# Autodesk Inventor assembly: SuspensionFinalShowdown
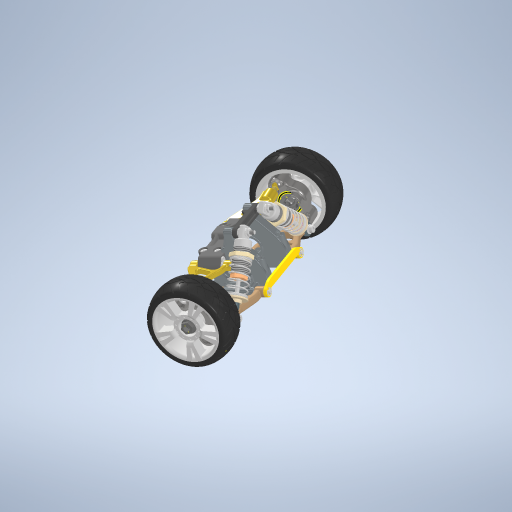
[picture p0: Inventor's stored thumbnail of the model, 512x512]
Saved by Autodesk Inventor 2024 (Build 280153000, 153)
## iProperties
Created: 2023-07-07
Part Number: SuspensionFinalShowdown
Document SubType Name: Assembly
Designer: birud
Author: birud
## Documents named in this file (20)
- C:\Users\_Astitva_Aryan_\Downloads\ES101_Components_Group5\Suspension_Final_Assembly.iam
- C:\Users\_Astitva_Aryan_\Downloads\ES101_Components_Group5\Components_derived\Front side plate L-1.ipt
- C:\Users\_Astitva_Aryan_\Downloads\ES101_Components_Group5\Components_derived\Front side plate R-1.ipt
- C:\Users\_Astitva_Aryan_\Downloads\ES101_Components_Group5\Components_derived\Front upper mount.ipt
- C:\Users\_Astitva_Aryan_\Downloads\ES101_Components_Group5\Components_derived\Front Shock Brace-1.ipt
- C:\Users\_Astitva_Aryan_\Downloads\ES101_Components_Group5\Components_derived\Front Lower arm Brace.ipt
- C:\Users\_Astitva_Aryan_\Downloads\ES101_Components_Group5\Components_derived\Front Lower Hinge Pin.ipt
- C:\Users\_Astitva_Aryan_\Downloads\ES101_Components_Group5\Components_derived\Front Upper Hinge Pin.ipt
- C:\Users\_Astitva_Aryan_\Downloads\ES101_Components_Group5\Components_derived\Front Upper Arm with pillow ball.iam
- C:\Users\_Astitva_Aryan_\Downloads\ES101_Components_Group5\Components_derived\Front Lower Arm with pillow ball.iam
- C:\Users\_Astitva_Aryan_\Downloads\ES101_Components_Group5\Components_derived\Shock Bushing.ipt
- C:\Users\_Astitva_Aryan_\Downloads\ES101_Components_Group5\Components_derived\Front Suspension Adjustment Clip.ipt
- C:\Users\_Astitva_Aryan_\Downloads\ES101_Components_Group5\Components_derived\a shock absorber.iam
- C:\Users\_Astitva_Aryan_\Downloads\ES101_Components_Group5\Components_derived\Front Hub Carrier L.iam
- C:\Users\_Astitva_Aryan_\Downloads\ES101_Components_Group5\Components_derived\SA E-Clip.ipt
- C:\Users\_Astitva_Aryan_\Downloads\ES101_Components_Group5\Components_derived\ANSI B18.22.1 - No. 5.ipt
- C:\Users\_Astitva_Aryan_\Downloads\ES101_Components_Group5\Components_derived\P12.ipt
- C:\Users\_Astitva_Aryan_\Downloads\ES101_Components_Group5\Components_derived\P20.ipt
- C:\Users\_Astitva_Aryan_\Downloads\ES101_Components_Group5\Components_derived\P20-nut.ipt
- C:\Users\_Astitva_Aryan_\Downloads\ES101_Components_Group5\Components_derived\Front Hub Carrier R.iam
## Components (43 placed, 19 different names)
1. Front side plate L-1:1 — Mate:1, Flush:1, Mate:2, Mate:4, Mate:5, Mate:6, Mate:7, Mate:12, Mate:50, Mate:52, Insert:11
2. Front side plate R-1:1 — Mate:1, Flush:1, Mate:2, Mate:3, Mate:8, Mate:9, Mate:11, Mate:21, Mate:22, Insert:12
3. Front upper mount:1 — Mate:3, Mate:4, Mate:5, Mate:14, Mate:15, Mate:24, Mate:26, Mate:42, Mate:47, Mate:48, Insert:5, Insert:6, Insert:7, Insert:8
4. Front Shock Brace-1:1 — Mate:6, Mate:7, Mate:8, Mate:17, Mate:18, Mate:19, Mate:20
5. Front Lower arm Brace:1 — Mate:9, Flush:4, Mate:51
6. Front Lower Hinge Pin:1 — Mate:12, Flush:2, Mate:49
7. Front Lower Hinge Pin:2 — Mate:11, Flush:2, Mate:33, Mate:34, Flush:4, Mate:35
8. Front Upper Hinge Pin:1 — Mate:15, Flush:3, Mate:23, Mate:37, Mate:38, Flush:5, Mate:39, Mate:40
9. Front Upper Hinge Pin:2 — Mate:14, Flush:3, Mate:41, Mate:43, Mate:44, Mate:45
10. Front Lower Arm with pillow ball:1 [sub-assembly] — Mate:21, Mate:22, Mate:29, Mate:32, Mate:36
11. Shock Bushing:1 — Mate:17, Mate:18, Mate:28, Mate:30, Insert:2
12. Shock Bushing:2 — Mate:19, Mate:20, Mate:56, Mate:58, Insert:4
13. Front Upper Arm with pillow ball:1 [sub-assembly] — Mate:23, Mate:24, Mate:27, Mate:31, Flush:5
14. Front Suspension Adjustment Clip:1 — Mate:26, Mate:27
15. a shock absorber:1 [sub-assembly] — Mate:28, Mate:29, Mate:30, Insert:1, Insert:10
16. Front Hub Carrier L:1 [sub-assembly] — Mate:31, Mate:32
17. SA E-Clip:1 — Mate:33, Mate:34
18. SA E-Clip:2 — Mate:35, Mate:36
19. SA E-Clip:3 — Mate:37, Mate:38
20. SA E-Clip:4 — Mate:39, Mate:40
21. ANSI B18.22.1 - No. 5:1 — Insert:1
22. ANSI B18.22.1 - No. 5:2 — Insert:2, Mate:60
23. Front Upper Arm with pillow ball:2 [sub-assembly] — Mate:41, Mate:42, Mate:46, Mate:63
24. SA E-Clip:5 — Mate:43, Mate:44
25. SA E-Clip:6 — Mate:45, Mate:46
26. Front Suspension Adjustment Clip:2 — Mate:47, Mate:48
27. Front Lower Arm with pillow ball:2 [sub-assembly] — Mate:49, Mate:50, Mate:54, Mate:55, Mate:57, Mate:64
28. SA E-Clip:7 — Mate:51, Mate:52
29. SA E-Clip:8 — Mate:54, Mate:55
30. a shock absorber:2 [sub-assembly] — Mate:56, Mate:57, Mate:58, Insert:3, Insert:9
31. ANSI B18.22.1 - No. 5:3 — Insert:3
32. ANSI B18.22.1 - No. 5:4 — Insert:4, Mate:61
33. P12:1 — Insert:5
34. P12:2 — Insert:8
35. P12:3 — Insert:7
36. P12:4 — Insert:6
37. P12:5 — Insert:9
38. P12:6 — Insert:10
39. P20:1 — Insert:12, Mate:59
40. P20:2 — Insert:11, Mate:62
41. P20-nut:1 — Mate:59, Mate:60
42. P20-nut:2 — Mate:61, Mate:62
43. Front Hub Carrier R:1 [sub-assembly] — Mate:63, Mate:64
## Relationships (76: Mate 59, Insert 12, Flush 5)
- Mate:1: Front side plate L-1:1 ↔ Front side plate R-1:1
- Flush:1: Front side plate L-1:1 ↔ Front side plate R-1:1
- Mate:2 (251.46 mm): Front side plate L-1:1 ↔ Front side plate R-1:1
- Mate:3: Front side plate R-1:1 ↔ Front upper mount:1
- Mate:4: Front side plate L-1:1 ↔ Front upper mount:1
- Mate:5: Front side plate L-1:1 ↔ Front upper mount:1
- Mate:6: Front side plate L-1:1 ↔ Front Shock Brace-1:1
- Mate:7: Front side plate L-1:1 ↔ Front Shock Brace-1:1
- Mate:8: Front side plate R-1:1 ↔ Front Shock Brace-1:1
- Mate:9: Front side plate R-1:1 ↔ Front Lower arm Brace:1
- Mate:11: Front side plate R-1:1 ↔ Front Lower Hinge Pin:2
- Mate:12: Front side plate L-1:1 ↔ Front Lower Hinge Pin:1
- Flush:2: Front Lower Hinge Pin:1 ↔ Front Lower Hinge Pin:2
- Mate:14: Front upper mount:1 ↔ Front Upper Hinge Pin:2
- Mate:15: Front upper mount:1 ↔ Front Upper Hinge Pin:1
- Flush:3: Front Upper Hinge Pin:1 ↔ Front Upper Hinge Pin:2
- Mate:17: Front Shock Brace-1:1 ↔ Shock Bushing:1
- Mate:18: Front Shock Brace-1:1 ↔ Shock Bushing:1
- Mate:19: Front Shock Brace-1:1 ↔ Shock Bushing:2
- Mate:20: Front Shock Brace-1:1 ↔ Shock Bushing:2
- Mate:21: Front side plate R-1:1 ↔ Front Lower Arm with pillow ball:1
- Mate:22: Front side plate R-1:1 ↔ Front Lower Arm with pillow ball:1
- Mate:23: Front Upper Hinge Pin:1 ↔ Front Upper Arm with pillow ball:1
- Mate:24: Front upper mount:1 ↔ Front Upper Arm with pillow ball:1
- Mate:26: Front upper mount:1 ↔ Front Suspension Adjustment Clip:1
- Mate:27: Front Upper Arm with pillow ball:1 ↔ Front Suspension Adjustment Clip:1
- Mate:28: Shock Bushing:1 ↔ a shock absorber:1
- Mate:29: Front Lower Arm with pillow ball:1 ↔ a shock absorber:1
- Mate:30: Shock Bushing:1 ↔ a shock absorber:1
- Mate:31: Front Upper Arm with pillow ball:1 ↔ Front Hub Carrier L:1
- Mate:32: Front Lower Arm with pillow ball:1 ↔ Front Hub Carrier L:1
- Mate:33: Front Lower Hinge Pin:2 ↔ SA E-Clip:1
- Mate:34: Front Lower Hinge Pin:2 ↔ SA E-Clip:1
- Flush:4: Front Lower arm Brace:1 ↔ Front Lower Hinge Pin:2
- Mate:35: Front Lower Hinge Pin:2 ↔ SA E-Clip:2
- Mate:36: Front Lower Arm with pillow ball:1 ↔ SA E-Clip:2
- Mate:37: Front Upper Hinge Pin:1 ↔ SA E-Clip:3
- Mate:38: Front Upper Hinge Pin:1 ↔ SA E-Clip:3
- Flush:5: Front Upper Hinge Pin:1 ↔ Front Upper Arm with pillow ball:1
- Mate:39: Front Upper Hinge Pin:1 ↔ SA E-Clip:4
- Mate:40: Front Upper Hinge Pin:1 ↔ SA E-Clip:4
- Insert:1: a shock absorber:1 ↔ ANSI B18.22.1 - No. 5:1
- Insert:2: Shock Bushing:1 ↔ ANSI B18.22.1 - No. 5:2
- Mate:41: Front Upper Hinge Pin:2 ↔ Front Upper Arm with pillow ball:2
- Mate:42: Front upper mount:1 ↔ Front Upper Arm with pillow ball:2
- Mate:43: Front Upper Hinge Pin:2 ↔ SA E-Clip:5
- Mate:44: Front Upper Hinge Pin:2 ↔ SA E-Clip:5
- Mate:45: Front Upper Hinge Pin:2 ↔ SA E-Clip:6
- Mate:46: Front Upper Arm with pillow ball:2 ↔ SA E-Clip:6
- Mate:47: Front upper mount:1 ↔ Front Suspension Adjustment Clip:2
- Mate:48: Front upper mount:1 ↔ Front Suspension Adjustment Clip:2
- Mate:49: Front Lower Hinge Pin:1 ↔ Front Lower Arm with pillow ball:2
- Mate:50: Front side plate L-1:1 ↔ Front Lower Arm with pillow ball:2
- Mate:51: Front Lower arm Brace:1 ↔ SA E-Clip:7
- Mate:52: Front side plate L-1:1 ↔ SA E-Clip:7
- Mate:54: Front Lower Arm with pillow ball:2 ↔ SA E-Clip:8
- Mate:55: Front Lower Arm with pillow ball:2 ↔ SA E-Clip:8
- Mate:56: Shock Bushing:2 ↔ a shock absorber:2
- Mate:57: Front Lower Arm with pillow ball:2 ↔ a shock absorber:2
- Mate:58: Shock Bushing:2 ↔ a shock absorber:2
- Insert:3: a shock absorber:2 ↔ ANSI B18.22.1 - No. 5:3
- Insert:4: Shock Bushing:2 ↔ ANSI B18.22.1 - No. 5:4
- Insert:5: Front upper mount:1 ↔ P12:1
- Insert:6: Front upper mount:1 ↔ P12:4
- Insert:7: Front upper mount:1 ↔ P12:3
- Insert:8: Front upper mount:1 ↔ P12:2
- Insert:9: a shock absorber:2 ↔ P12:5
- Insert:10: a shock absorber:1 ↔ P12:6
- Insert:11: Front side plate L-1:1 ↔ P20:2
- Insert:12: Front side plate R-1:1 ↔ P20:1
- Mate:59: P20:1 ↔ P20-nut:1
- Mate:60: ANSI B18.22.1 - No. 5:2 ↔ P20-nut:1
- Mate:61: ANSI B18.22.1 - No. 5:4 ↔ P20-nut:2
- Mate:62: P20:2 ↔ P20-nut:2
- Mate:63: Front Upper Arm with pillow ball:2 ↔ Front Hub Carrier R:1
- Mate:64: Front Lower Arm with pillow ball:2 ↔ Front Hub Carrier R:1
